# Autodesk Inventor assembly: Assembly1
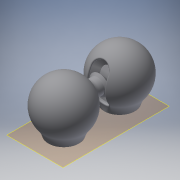
[picture p0: Inventor's stored thumbnail of the model, 180x180]
Saved by Autodesk Inventor 2017 (Build 210142000, 142)
## iProperties
Created: 2017-02-21
Part Number: Assembly1
Document SubType Name: Assembly
Designer: PLTW
Author: PLTW
## Documents named in this file (3)
- C:\Users\ellie\Documents\Inventor\Tea Cat\Assembly1.iam
- C:\Users\ellie\Documents\Inventor\Tea Cat\Body.ipt
- C:\Users\ellie\Documents\Inventor\Tea Cat\The Thing.ipt
## Components (2 placed, 2 different names)
1. Body:1 — Flush:1
2. The Thing:1 — Flush:1
## Relationships (1: Flush 1)
- Flush:1: Body:1 ↔ The Thing:1
